# Autodesk Inventor assembly: Wheel Orientation
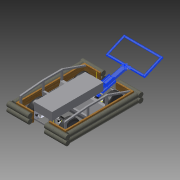
[picture p0: Inventor's stored thumbnail of the model, 180x180]
Saved by Autodesk Inventor 2015 (Build 190159000, 159)
## iProperties
Created: 2016-01-19
Part Number: Wheel Orientation
Document SubType Name: Assembly
Designer: sethbattis
Author: sethbattis
## Documents named in this file (12)
- \\area51\team3566\cad\FRC 2016\Space Claims.iam
- \\area51\team3566\cad\FRC 2016\Snow Blower Tire with Gear Box and Mini-CIM.iam
- \\area51\team3566\cad\FRC 2016\Side Bumper.ipt
- \\area51\team3566\cad\FRC 2016\Catapult Base.ipt
- \\area51\team3566\cad\FRC 2016\Chassis.ipt
- \\area51\team3566\cad\FRC 2016\Top Axle.ipt
- \\area51\team3566\cad\FRC 2016\Snow Blower Tire with Gear Box and Mini-CIM_MIR1.iam
- \\area51\team3566\cad\FRC 2016\Snow Blower Tire with Gear Box and Mini-CIM_MIR3.iam
- \\area51\team3566\cad\FRC 2016\Top Axle_MIR1.ipt
- \\area51\team3566\cad\FRC 2016\Snow Blower Tire with Gear Box and Mini-CIM_MIR1_MIR1.iam
- \\area51\team3566\cad\FRC 2016\Bread Pan.ipt
- \\area51\team3566\cad\FRC 2016\Ball Picker Upper.iam
## Components (12 placed, 11 different names)
1. Chassis:1 — Mate:25, Mate:26, Mate:29, Mate:30, Mate:31, Mate:32, Mate:33, Mate:34, Mate:35, Mate:36, Mate:39, Mate:40, Mate:41, Mate:42, Mate:43, Flush:1, Mate:44, Mate:47
2. Catapult Base:1 — Mate:35, Mate:36
3. Bread Pan:1 — Mate:42, Mate:43, Flush:1
4. Ball Picker Upper:1 [sub-assembly] — Mate:45, Mate:46, Mate:47
5. Top Axle:1 — Mate:25, Mate:26, Mate:39, Rotational:1, Rotational:2, Mate:45, Mate:46
6. Snow Blower Tire with Gear Box and Mini-CIM:1 [sub-assembly] — Rotational:1
7. Snow Blower Tire with Gear Box and Mini-CIM_MIR1:1 [sub-assembly] — Rotational:2
8. Snow Blower Tire with Gear Box and Mini-CIM_MIR3:1 [sub-assembly] — Rotational:3
9. Top Axle_MIR1:1 — Rotational:3, Rotational:4, Mate:40, Mate:41, Mate:44
10. Snow Blower Tire with Gear Box and Mini-CIM_MIR1_MIR1:1 [sub-assembly] — Rotational:4
11. Side Bumper:2 — Mate:32, Mate:33, Mate:34
12. Side Bumper:1 — Mate:29, Mate:30, Mate:31
## Relationships (24: Mate 19, RevoluteJoint 4, Flush 1)
- Mate:25: Chassis:1 ↔ Top Axle:1
- Mate:26: Chassis:1 ↔ Top Axle:1
- Mate:29: Chassis:1 ↔ Side Bumper:1
- Mate:30: Chassis:1 ↔ Side Bumper:1
- Mate:31: Chassis:1 ↔ Side Bumper:1
- Mate:32: Chassis:1 ↔ Side Bumper:2
- Mate:33: Chassis:1 ↔ Side Bumper:2
- Mate:34: Chassis:1 ↔ Side Bumper:2
- Mate:35: Chassis:1 ↔ Catapult Base:1
- Mate:36: Chassis:1 ↔ Catapult Base:1
- Mate:39: Chassis:1 ↔ Top Axle:1
- Rotational:1 [RevoluteJoint]: Top Axle:1 ↔ Snow Blower Tire with Gear Box and Mini-CIM:1
- Rotational:2 [RevoluteJoint]: Top Axle:1 ↔ Snow Blower Tire with Gear Box and Mini-CIM_MIR1:1
- Rotational:3 [RevoluteJoint]: Snow Blower Tire with Gear Box and Mini-CIM_MIR3:1 ↔ Top Axle_MIR1:1
- Rotational:4 [RevoluteJoint]: Top Axle_MIR1:1 ↔ Snow Blower Tire with Gear Box and Mini-CIM_MIR1_MIR1:1
- Mate:40: Chassis:1 ↔ Top Axle_MIR1:1
- Mate:41: Chassis:1 ↔ Top Axle_MIR1:1
- Mate:42: Chassis:1 ↔ Bread Pan:1
- Mate:43: Chassis:1 ↔ Bread Pan:1
- Flush:1: Chassis:1 ↔ Bread Pan:1
- Mate:44: Chassis:1 ↔ Top Axle_MIR1:1
- Mate:45: Ball Picker Upper:1 ↔ Top Axle:1
- Mate:46: Ball Picker Upper:1 ↔ Top Axle:1
- Mate:47: Chassis:1 ↔ Ball Picker Upper:1
